# Autodesk Inventor assembly: Full_Design
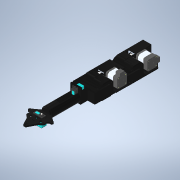
[picture p0: Inventor's stored thumbnail of the model, 180x180]
Saved by Autodesk Inventor 2022 (Build 260153000, 153)
## iProperties
Created: 2022-02-25
Part Number: Full_Design
Document SubType Name: Assembly
Designer: Mlees
Author: Mlees
## Documents named in this file (28)
- C:\Users\Mlees\Desktop\504Engineering\Stepper-Servo_Based_Robotic_Arm\Designs\Version_7\Full_Design.iam
- C:\Users\Mlees\Desktop\504Engineering\Stepper-Servo_Based_Robotic_Arm\Designs\Version_7\Created_Parts\24_Teeth_Sun_Gear.ipt
- C:\Users\Mlees\Desktop\504Engineering\Stepper-Servo_Based_Robotic_Arm\Designs\Version_7\Created_Parts\36_Teeth_Planet_Gear.ipt
- C:\Users\Mlees\Desktop\504Engineering\Stepper-Servo_Based_Robotic_Arm\Designs\Version_7\Created_Parts\Joint1.ipt
- C:\Users\Mlees\Desktop\504Engineering\Stepper-Servo_Based_Robotic_Arm\Designs\Version_7\Created_Parts\Plamet_Carrier.ipt
- C:\Users\Mlees\Desktop\504Engineering\Stepper-Servo_Based_Robotic_Arm\Designs\Version_7\Created_Parts\Planet_Carrier_Modifed_with_sun_gear.ipt
- C:\Users\Mlees\Desktop\504Engineering\Stepper-Servo_Based_Robotic_Arm\Designs\Version_7\Created_Parts\Gear_Cover_modified.ipt
- C:\Users\Mlees\Desktop\504Engineering\Stepper-Servo_Based_Robotic_Arm\Designs\Version_7\Created_Parts\Combined_Gear_Box_Modified_2.ipt
- C:\Users\Mlees\Desktop\504Engineering\Stepper-Servo_Based_Robotic_Arm\Designs\Version_7\Downloaded_Parts\GT2 20T Drive Pulley.ipt
- C:\Users\Mlees\Desktop\504Engineering\Stepper-Servo_Based_Robotic_Arm\Designs\Version_7\Downloaded_Parts\GT2 60T Drive Pulley.ipt
- C:\Users\Mlees\Desktop\504Engineering\Stepper-Servo_Based_Robotic_Arm\Designs\Version_7\Downloaded_Parts\9403T15_Tight-Tolerance High-Strength 7075 Aluminum Rod.ipt
- C:\Users\Mlees\Desktop\504Engineering\Stepper-Servo_Based_Robotic_Arm\Designs\Version_7\Downloaded_Parts\124125202-9-stp-mtr-17040w\stp-mtr-17040w.ipt
- C:\Users\Mlees\Desktop\504Engineering\Stepper-Servo_Based_Robotic_Arm\Designs\Version_7\Created_Parts\Combined_Gear_Box_Modified_3.ipt
- C:\Users\Mlees\Desktop\504Engineering\Stepper-Servo_Based_Robotic_Arm\Designs\Version_7\Downloaded_Parts\uploads_files_140274_ServoSW-1211SG.ipt
- C:\Users\Mlees\Desktop\504Engineering\Stepper-Servo_Based_Robotic_Arm\Designs\Version_7\Created_Parts\Metal_AttachmentBracket.ipt
- C:\Users\Mlees\Desktop\504Engineering\Stepper-Servo_Based_Robotic_Arm\Designs\Version_7\Created_Parts\Tilt_Bracket_Output_2.ipt
- C:\Users\Mlees\Desktop\504Engineering\Stepper-Servo_Based_Robotic_Arm\Designs\Version_7\Created_Parts\Belt_Bearing_Holder.ipt
- C:\Users\Mlees\Desktop\504Engineering\Stepper-Servo_Based_Robotic_Arm\Designs\Version_7\Created_Parts\Belt_Bearing_Holder_p2.ipt
- C:\Users\Mlees\Desktop\504Engineering\Stepper-Servo_Based_Robotic_Arm\Designs\Version_7\Created_Parts\Belt_Tension_Bearing.ipt
- C:\Users\Mlees\Desktop\504Engineering\Stepper-Servo_Based_Robotic_Arm\Designs\Version_7\Created_Parts\Twist_Attachment_To_Servo_Horn.ipt
- C:\Users\Mlees\Desktop\504Engineering\Stepper-Servo_Based_Robotic_Arm\Designs\Version_7\Created_Parts\Twist_Servo_Horn.ipt
- C:\Users\Mlees\Desktop\504Engineering\Stepper-Servo_Based_Robotic_Arm\Designs\Version_7\Created_Parts\Twist_Rod.ipt
- C:\Users\Mlees\Desktop\504Engineering\Stepper-Servo_Based_Robotic_Arm\Designs\Version_7\Created_Parts\Tilt_Bracket_Output_2_Lid.ipt
- C:\Users\Mlees\Desktop\504Engineering\Stepper-Servo_Based_Robotic_Arm\Designs\Version_7\Created_Parts\Claw_Attachment.ipt
- C:\Users\Mlees\Desktop\504Engineering\Stepper-Servo_Based_Robotic_Arm\Designs\Version_7\Created_Parts\Mag_Shield_Back.ipt
- C:\Users\Mlees\Desktop\504Engineering\Stepper-Servo_Based_Robotic_Arm\Designs\Version_8\Created_Parts\Bearing_Side_Tilt.ipt
- C:\Users\Mlees\Desktop\504Engineering\Stepper-Servo_Based_Robotic_Arm\Designs\Version_8\Created_Parts\Claw_Finger.ipt
- C:\Users\Mlees\Desktop\504Engineering\Stepper-Servo_Based_Robotic_Arm\Designs\Version_8\Created_Parts\Claw_Main.ipt
## Components (57 placed, 27 different names)
1. 24_Teeth_Sun_Gear:1 — Rigid:11, Rotational:15, Rotation:4
2. 36_Teeth_Planet_Gear:1 — Mate:11
3. 36_Teeth_Planet_Gear:2 — Mate:12
4. 36_Teeth_Planet_Gear:3 — Mate:10
5. 36_Teeth_Planet_Gear:4 — Mate:8
6. 36_Teeth_Planet_Gear:5 — Mate:9
7. 36_Teeth_Planet_Gear:6 — Mate:7
8. Joint1:1 — Mate:18, Mate:19, Mate:20, Mate:21, Mate:22, Mate:23, Mate:24, Flush:5, Mate:25, Rotational:13, Mate:32, Mate:33, Flush:6, Rigid:12
9. Plamet_Carrier:1 — Mate:10, Mate:11, Mate:12, Rotational:8, Rotation:2, Mate:19, Mate:20
10. Planet_Carrier_Modifed_with_sun_gear:1 — Mate:7, Mate:8, Mate:9, Rotational:7, Rotation:1, Rotational:8, Rotation:2
11. Gear_Cover_modified:1 — Mate:13, Flush:2, Flush:3, Mate:18
12. Combined_Gear_Box_Modified_2:1 — Rotational:6, Mate:4, Mate:5, Mate:6, Mate:13, Flush:2, Flush:3
13. GT2 20T Drive Pulley:1 — Rotational:9
14. GT2 60T Drive Pulley:1 — Rotational:14, Rigid:10
15. 9403T15_Tight-Tolerance High-Strength 7075 Aluminum Rod:1 — Rigid:8, Rigid:1, Rotation:1
16. stp-mtr-17040w:1 — Mate:3, Rotational:1
17. stp-mtr-17040w:2 — Rigid:9, Rotational:9
18. Combined_Gear_Box_Modified_2:2 — Rotational:14, Mate:32, Mate:33, Flush:6, Mate:34, Flush:7, Flush:8
19. Combined_Gear_Box_Modified_3:1 — Mate:1, Flush:1, Mate:2, Rotational:2, Mate:4, Mate:5, Mate:6, Mate:14, Mate:15, Mate:16, Mate:17, Flush:4
20. GT2 20T Drive Pulley:2 — Rotational:1, Rotation:3
21. GT2 60T Drive Pulley:2 — Rotational:6, Rigid:8, Rotation:3
22. 9403T15_Tight-Tolerance High-Strength 7075 Aluminum Rod:2 — Rigid:10, Rigid:11
23. 24_Teeth_Sun_Gear:2 — Rigid:1, Rotational:7
24. 36_Teeth_Planet_Gear:7 — Mate:29
25. Plamet_Carrier:2 — Mate:29, Mate:30, Mate:31, Rotational:16, Rotation:5, Mate:36, Mate:37
26. Planet_Carrier_Modifed_with_sun_gear:2 — Mate:26, Mate:27, Mate:28, Rotational:15, Rotation:4, Rotational:16, Rotation:5
27. 36_Teeth_Planet_Gear:8 — Mate:31
28. 36_Teeth_Planet_Gear:9 — Mate:28
29. 36_Teeth_Planet_Gear:10 — Mate:26
30. 36_Teeth_Planet_Gear:11 — Mate:27
31. 36_Teeth_Planet_Gear:12 — Mate:30
32. Gear_Cover_modified:2 — Mate:34, Flush:7, Flush:8, Mate:35
33. Metal_AttachmentBracket:1 — Mate:1, Flush:1, Mate:2, Mate:3
34. Tilt_Bracket_Output_2:1 — Mate:35, Mate:36, Mate:37, Rigid:16, Rigid:17
35. Belt_Bearing_Holder:1 — Rotational:2, Rotational:3, Rotational:5
36. Belt_Bearing_Holder_p2:1 — Rotational:5
37. Belt_Tension_Bearing:1 — Rotational:3, Rotational:4
38. Belt_Tension_Bearing:3 — Rotational:4
39. uploads_files_140274_ServoSW-1211SG:1 — Rotational:17, Rigid:16
40. Twist_Attachment_To_Servo_Horn:1 — Rigid:13, Rigid:14
41. Twist_Servo_Horn:1 — Rotational:17, Rigid:13
42. Twist_Rod:1 — Rigid:14, Rigid:15
43. Tilt_Bracket_Output_2_Lid:1 — Rigid:17
44. Claw_Attachment:1 — Rigid:15, Rigid:18
45. Mag_Shield_Back:1 — Mate:21, Mate:22, Mate:23
46. Mag_Shield_Back:2 — Mate:14, Mate:15, Mate:16
47. Bearing_Side_Tilt:1 — Mate:17, Flush:4
48. Metal_AttachmentBracket:2 — Mate:24, Flush:5, Mate:25, Rigid:9
49. Belt_Bearing_Holder:2 — Rotational:13
50. Belt_Bearing_Holder_p2:2
51. Belt_Tension_Bearing:4
52. Belt_Tension_Bearing:5
53. Bearing_Side_Tilt:2 — Rigid:12
54. Claw_Finger:1 — Rigid:20
55. Claw_Main:1 — Rigid:18, Rigid:19, Rigid:20, Rigid:21
56. Claw_Finger:2 — Rigid:19
57. uploads_files_140274_ServoSW-1211SG:2 — Rigid:21
## Relationships (82: Mate 37, RevoluteJoint 17, WeldJoint 15, Flush 8, RelateRotation 5)
- Mate:1: Combined_Gear_Box_Modified_3:1 ↔ Metal_AttachmentBracket:1
- Flush:1: Combined_Gear_Box_Modified_3:1 ↔ Metal_AttachmentBracket:1
- Mate:2: Combined_Gear_Box_Modified_3:1 ↔ Metal_AttachmentBracket:1
- Mate:3: stp-mtr-17040w:1 ↔ Metal_AttachmentBracket:1
- Rotational:1 [RevoluteJoint] (5 mm): stp-mtr-17040w:1 ↔ GT2 20T Drive Pulley:2
- Rotational:2 [RevoluteJoint] (10 mm): Combined_Gear_Box_Modified_3:1 ↔ Belt_Bearing_Holder:1
- Rotational:3 [RevoluteJoint]: Belt_Bearing_Holder:1 ↔ Belt_Tension_Bearing:1
- Rotational:4 [RevoluteJoint]: Belt_Tension_Bearing:1 ↔ Belt_Tension_Bearing:3
- Rotational:5 [RevoluteJoint]: Belt_Bearing_Holder:1 ↔ Belt_Bearing_Holder_p2:1
- Rotational:6 [RevoluteJoint]: Combined_Gear_Box_Modified_2:1 ↔ GT2 60T Drive Pulley:2
- Rigid:8 [WeldJoint]: 9403T15_Tight-Tolerance High-Strength 7075 Aluminum Rod:1 ↔ GT2 60T Drive Pulley:2
- Rigid:1 [WeldJoint]: 9403T15_Tight-Tolerance High-Strength 7075 Aluminum Rod:1 ↔ 24_Teeth_Sun_Gear:2
- Mate:4: Combined_Gear_Box_Modified_2:1 ↔ Combined_Gear_Box_Modified_3:1
- Mate:5: Combined_Gear_Box_Modified_2:1 ↔ Combined_Gear_Box_Modified_3:1
- Mate:6: Combined_Gear_Box_Modified_2:1 ↔ Combined_Gear_Box_Modified_3:1
- Mate:7: 36_Teeth_Planet_Gear:6 ↔ Planet_Carrier_Modifed_with_sun_gear:1
- Mate:8: 36_Teeth_Planet_Gear:4 ↔ Planet_Carrier_Modifed_with_sun_gear:1
- Mate:9: 36_Teeth_Planet_Gear:5 ↔ Planet_Carrier_Modifed_with_sun_gear:1
- Rotational:7 [RevoluteJoint]: Planet_Carrier_Modifed_with_sun_gear:1 ↔ 24_Teeth_Sun_Gear:2
- Rotation:1 [RelateRotation] (5 ul): Planet_Carrier_Modifed_with_sun_gear:1 ↔ 9403T15_Tight-Tolerance High-Strength 7075 Aluminum Rod:1
- Mate:10: 36_Teeth_Planet_Gear:3 ↔ Plamet_Carrier:1
- Mate:11: 36_Teeth_Planet_Gear:1 ↔ Plamet_Carrier:1
- Mate:12: 36_Teeth_Planet_Gear:2 ↔ Plamet_Carrier:1
- Rotational:8 [RevoluteJoint]: Plamet_Carrier:1 ↔ Planet_Carrier_Modifed_with_sun_gear:1
- Rotation:2 [RelateRotation] (5 ul): Plamet_Carrier:1 ↔ Planet_Carrier_Modifed_with_sun_gear:1
- Rotation:3 [RelateRotation] (0.3333 ul): GT2 20T Drive Pulley:2 ↔ GT2 60T Drive Pulley:2
- Mate:13: Gear_Cover_modified:1 ↔ Combined_Gear_Box_Modified_2:1
- Flush:2: Gear_Cover_modified:1 ↔ Combined_Gear_Box_Modified_2:1
- Flush:3: Gear_Cover_modified:1 ↔ Combined_Gear_Box_Modified_2:1
- Mate:14: Combined_Gear_Box_Modified_3:1 ↔ Mag_Shield_Back:2
- Mate:15: Combined_Gear_Box_Modified_3:1 ↔ Mag_Shield_Back:2
- Mate:16: Combined_Gear_Box_Modified_3:1 ↔ Mag_Shield_Back:2
- Mate:17: Combined_Gear_Box_Modified_3:1 ↔ Bearing_Side_Tilt:1
- Flush:4: Combined_Gear_Box_Modified_3:1 ↔ Bearing_Side_Tilt:1
- Mate:18: Joint1:1 ↔ Gear_Cover_modified:1
- Mate:19: Joint1:1 ↔ Plamet_Carrier:1
- Mate:20: Joint1:1 ↔ Plamet_Carrier:1
- Mate:21: Joint1:1 ↔ Mag_Shield_Back:1
- Mate:22: Joint1:1 ↔ Mag_Shield_Back:1
- Mate:23: Joint1:1 ↔ Mag_Shield_Back:1
- Mate:24: Joint1:1 ↔ Metal_AttachmentBracket:2
- Flush:5: Joint1:1 ↔ Metal_AttachmentBracket:2
- Mate:25: Joint1:1 ↔ Metal_AttachmentBracket:2
- Rigid:9 [WeldJoint]: stp-mtr-17040w:2 ↔ Metal_AttachmentBracket:2
- Rotational:9 [RevoluteJoint] (5 mm): GT2 20T Drive Pulley:1 ↔ stp-mtr-17040w:2
- [RevoluteJoint]: Belt_Bearing_Holder:2 ↔ Belt_Tension_Bearing:4
- [RevoluteJoint]: Belt_Tension_Bearing:4 ↔ Belt_Tension_Bearing:5
- [RevoluteJoint]: Belt_Bearing_Holder:2 ↔ Belt_Bearing_Holder_p2:2
- Rotational:13 [RevoluteJoint] (10 mm): Joint1:1 ↔ Belt_Bearing_Holder:2
- Rotational:14 [RevoluteJoint]: GT2 60T Drive Pulley:1 ↔ Combined_Gear_Box_Modified_2:2
- Rigid:10 [WeldJoint]: GT2 60T Drive Pulley:1 ↔ 9403T15_Tight-Tolerance High-Strength 7075 Aluminum Rod:2
- Rigid:11 [WeldJoint]: 24_Teeth_Sun_Gear:1 ↔ 9403T15_Tight-Tolerance High-Strength 7075 Aluminum Rod:2
- Mate:26: Planet_Carrier_Modifed_with_sun_gear:2 ↔ 36_Teeth_Planet_Gear:10
- Mate:27: Planet_Carrier_Modifed_with_sun_gear:2 ↔ 36_Teeth_Planet_Gear:11
- Mate:28: Planet_Carrier_Modifed_with_sun_gear:2 ↔ 36_Teeth_Planet_Gear:9
- Rotational:15 [RevoluteJoint]: 24_Teeth_Sun_Gear:1 ↔ Planet_Carrier_Modifed_with_sun_gear:2
- Rotation:4 [RelateRotation] (5 ul): 24_Teeth_Sun_Gear:1 ↔ Planet_Carrier_Modifed_with_sun_gear:2
- Mate:29: 36_Teeth_Planet_Gear:7 ↔ Plamet_Carrier:2
- Mate:30: Plamet_Carrier:2 ↔ 36_Teeth_Planet_Gear:12
- Mate:31: Plamet_Carrier:2 ↔ 36_Teeth_Planet_Gear:8
- Rotational:16 [RevoluteJoint]: Plamet_Carrier:2 ↔ Planet_Carrier_Modifed_with_sun_gear:2
- Rotation:5 [RelateRotation] (5 ul): Plamet_Carrier:2 ↔ Planet_Carrier_Modifed_with_sun_gear:2
- Mate:32: Joint1:1 ↔ Combined_Gear_Box_Modified_2:2
- Mate:33: Joint1:1 ↔ Combined_Gear_Box_Modified_2:2
- Flush:6: Joint1:1 ↔ Combined_Gear_Box_Modified_2:2
- Mate:34: Combined_Gear_Box_Modified_2:2 ↔ Gear_Cover_modified:2
- Flush:7: Combined_Gear_Box_Modified_2:2 ↔ Gear_Cover_modified:2
- Flush:8: Combined_Gear_Box_Modified_2:2 ↔ Gear_Cover_modified:2
- Rigid:12 [WeldJoint]: Joint1:1 ↔ Bearing_Side_Tilt:2
- Mate:35: Gear_Cover_modified:2 ↔ Tilt_Bracket_Output_2:1
- Mate:36: Plamet_Carrier:2 ↔ Tilt_Bracket_Output_2:1
- Mate:37: Plamet_Carrier:2 ↔ Tilt_Bracket_Output_2:1
- Rotational:17 [RevoluteJoint]: uploads_files_140274_ServoSW-1211SG:1 ↔ Twist_Servo_Horn:1
- Rigid:13 [WeldJoint]: Twist_Attachment_To_Servo_Horn:1 ↔ Twist_Servo_Horn:1
- Rigid:14 [WeldJoint]: Twist_Attachment_To_Servo_Horn:1 ↔ Twist_Rod:1
- Rigid:15 [WeldJoint]: Twist_Rod:1 ↔ Claw_Attachment:1
- Rigid:16 [WeldJoint]: Tilt_Bracket_Output_2:1 ↔ uploads_files_140274_ServoSW-1211SG:1
- Rigid:17 [WeldJoint]: Tilt_Bracket_Output_2:1 ↔ Tilt_Bracket_Output_2_Lid:1
- Rigid:18 [WeldJoint]: Claw_Attachment:1 ↔ Claw_Main:1
- Rigid:19 [WeldJoint]: Claw_Main:1 ↔ Claw_Finger:2
- Rigid:20 [WeldJoint]: Claw_Finger:1 ↔ Claw_Main:1
- Rigid:21 [WeldJoint]: Claw_Main:1 ↔ uploads_files_140274_ServoSW-1211SG:2
## Named parameters: d202_d143 = 0 mm, d203_d144 = -179.614976 deg, d204_d145 = 0 mm, d205_d146 = -0.00516 deg, d206_d147 = 0 mm, d207_d148 = -179.61537 deg
